# Autodesk Inventor assembly: Ensamblaje2
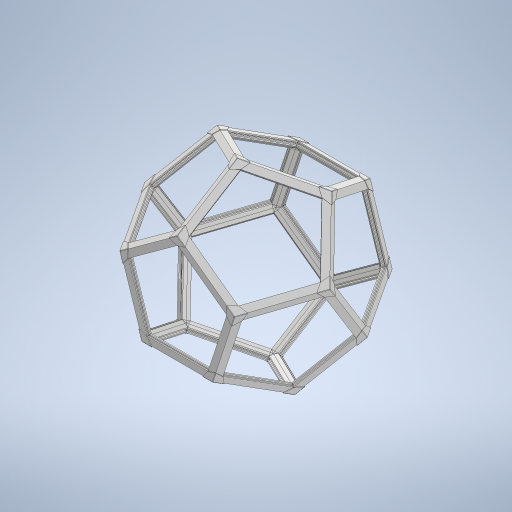
[picture p0: Inventor's stored thumbnail of the model, 512x512]
Saved by Autodesk Inventor 2024 (Build 280153000, 153)
## iProperties
Created: 2025-08-12
Part Number: Ensamblaje2
Document SubType Name: Assembly
Designer: sergi
Author: sergi
## Documents named in this file (3)
- C:\Users\sergi\OneDrive\Escritorio\Ensamblaje2.iam
- C:\Users\sergi\OneDrive\Escritorio\Ensamblaje1.iam
- C:\Users\sergi\OneDrive\Escritorio\Pieza1.ipt
## Components (52 placed, 2 different names)
1. Ensamblaje1:1 [sub-assembly] — Coincidencia:1, Coincidencia:2, Coincidencia:3, Coincidencia:4, Coincidencia:5, Coincidencia:6, Coincidencia:7, Coincidencia:8, Coincidencia:18
2. Pieza1:1 — Coincidencia:1, Coincidencia:2, Coincidencia:3, Coincidencia:15, Coincidencia:16, Coincidencia:17
3. Pieza1:2 — Coincidencia:4, Coincidencia:5, Coincidencia:12, Coincidencia:13, Coincidencia:14, Coincidencia:18
4. Pieza1:3 — Coincidencia:6, Coincidencia:7, Coincidencia:8, Coincidencia:9, Coincidencia:10, Coincidencia:11
5. Ensamblaje1:2 [sub-assembly] — Coincidencia:15, Coincidencia:16, Coincidencia:17, Coincidencia:28, Coincidencia:29, Coincidencia:30, Coincidencia:40, Coincidencia:41, Coincidencia:42
6. Ensamblaje1:3 [sub-assembly] — Coincidencia:9, Coincidencia:10, Coincidencia:11, Coincidencia:52, Coincidencia:53, Coincidencia:54, Coincidencia:64, Coincidencia:65, Coincidencia:66
7. Ensamblaje1:4 [sub-assembly] — Coincidencia:12, Coincidencia:13, Coincidencia:14, Coincidencia:76, Coincidencia:77, Coincidencia:78, Coincidencia:79, Coincidencia:80, Coincidencia:81
8. Ensamblaje1:5 [sub-assembly]
9. Pieza1:4 — Coincidencia:28, Coincidencia:29, Coincidencia:30
10. Pieza1:5
11. Pieza1:6 — Coincidencia:85, Coincidencia:86, Coincidencia:87
12. Ensamblaje1:6 [sub-assembly]
13. Pieza1:7
14. Pieza1:8 — Coincidencia:142, Coincidencia:143, Coincidencia:144
15. Pieza1:9 — Coincidencia:40, Coincidencia:41, Coincidencia:42
16. Ensamblaje1:7 [sub-assembly]
17. Pieza1:11 — Coincidencia:52, Coincidencia:53, Coincidencia:54
18. Pieza1:12
19. Ensamblaje1:8 [sub-assembly]
20. Pieza1:13 — Coincidencia:64, Coincidencia:65, Coincidencia:66
21. Pieza1:14
22. Pieza1:15 — Coincidencia:118, Coincidencia:119, Coincidencia:120
23. Ensamblaje1:9 [sub-assembly]
24. Pieza1:16 — Coincidencia:76, Coincidencia:77, Coincidencia:78
25. Pieza1:17 — Coincidencia:94, Coincidencia:95, Coincidencia:96
26. Pieza1:18 — Coincidencia:79, Coincidencia:80, Coincidencia:81
27. Ensamblaje1:10 [sub-assembly] — Coincidencia:85, Coincidencia:86, Coincidencia:87
28. Pieza1:19
29. Ensamblaje1:11 [sub-assembly] — Coincidencia:103, Coincidencia:104, Coincidencia:105
30. Ensamblaje1:12 [sub-assembly] — Coincidencia:94, Coincidencia:95, Coincidencia:96, Coincidencia:115, Coincidencia:116, Coincidencia:117
31. Pieza1:20
32. Pieza1:22 — Coincidencia:103, Coincidencia:104, Coincidencia:105, Coincidencia:145, Coincidencia:146, Coincidencia:147
33. Ensamblaje1:13 [sub-assembly]
34. Pieza1:23
35. Pieza1:24 — Coincidencia:115, Coincidencia:116, Coincidencia:117
36. Pieza1:25
37. Ensamblaje1:14 [sub-assembly] — Coincidencia:118, Coincidencia:119, Coincidencia:120, Coincidencia:124, Coincidencia:125, Coincidencia:126
38. Ensamblaje1:15 [sub-assembly] — Coincidencia:163, Coincidencia:164, Coincidencia:165
39. Pieza1:26 — Coincidencia:124, Coincidencia:125, Coincidencia:126
40. Ensamblaje1:16 [sub-assembly] — Coincidencia:142, Coincidencia:143, Coincidencia:144, Coincidencia:157, Coincidencia:158, Coincidencia:159
41. Pieza1:27
42. Ensamblaje1:17 [sub-assembly]
43. Ensamblaje1:18 [sub-assembly]
44. Pieza1:28
45. Pieza1:29
46. Ensamblaje1:19 [sub-assembly] — Coincidencia:145, Coincidencia:146, Coincidencia:147, Coincidencia:148, Coincidencia:149, Coincidencia:150
47. Pieza1:30 — Coincidencia:148, Coincidencia:149, Coincidencia:150, Coincidencia:151, Coincidencia:152, Coincidencia:153
48. Ensamblaje1:20 [sub-assembly] — Coincidencia:151, Coincidencia:152, Coincidencia:153
49. Pieza1:31 — Coincidencia:157, Coincidencia:158, Coincidencia:159
50. Ensamblaje1:21 [sub-assembly] — Coincidencia:160, Coincidencia:161, Coincidencia:162
51. Pieza1:32 — Coincidencia:160, Coincidencia:161, Coincidencia:162
52. Pieza1:33 — Coincidencia:163, Coincidencia:164, Coincidencia:165
## Relationships (153: Mate 153)
- Coincidencia:1 [Mate]: Ensamblaje1:1 ↔ Pieza1:1
- Coincidencia:2 [Mate]: Ensamblaje1:1 ↔ Pieza1:1
- Coincidencia:3 [Mate]: Ensamblaje1:1 ↔ Pieza1:1
- Coincidencia:4 [Mate]: Ensamblaje1:1 ↔ Pieza1:2
- Coincidencia:5 [Mate]: Ensamblaje1:1 ↔ Pieza1:2
- Coincidencia:6 [Mate]: Ensamblaje1:1 ↔ Pieza1:3
- Coincidencia:7 [Mate]: Ensamblaje1:1 ↔ Pieza1:3
- Coincidencia:8 [Mate]: Ensamblaje1:1 ↔ Pieza1:3
- Coincidencia:9 [Mate]: Pieza1:3 ↔ Ensamblaje1:3
- Coincidencia:10 [Mate]: Pieza1:3 ↔ Ensamblaje1:3
- Coincidencia:11 [Mate]: Pieza1:3 ↔ Ensamblaje1:3
- Coincidencia:12 [Mate]: Pieza1:2 ↔ Ensamblaje1:4
- Coincidencia:13 [Mate]: Pieza1:2 ↔ Ensamblaje1:4
- Coincidencia:14 [Mate]: Pieza1:2 ↔ Ensamblaje1:4
- Coincidencia:15 [Mate]: Pieza1:1 ↔ Ensamblaje1:2
- Coincidencia:16 [Mate]: Pieza1:1 ↔ Ensamblaje1:2
- Coincidencia:17 [Mate]: Pieza1:1 ↔ Ensamblaje1:2
- Coincidencia:18 [Mate]: Ensamblaje1:1 ↔ Pieza1:2
- [Mate]: Ensamblaje1:5 ↔ Pieza1:4
- [Mate]: Ensamblaje1:5 ↔ Pieza1:4
- [Mate]: Ensamblaje1:5 ↔ Pieza1:4
- [Mate]: Ensamblaje1:5 ↔ Pieza1:5
- [Mate]: Ensamblaje1:5 ↔ Pieza1:5
- [Mate]: Ensamblaje1:5 ↔ Pieza1:6
- [Mate]: Ensamblaje1:5 ↔ Pieza1:6
- [Mate]: Ensamblaje1:5 ↔ Pieza1:6
- [Mate]: Ensamblaje1:5 ↔ Pieza1:5
- Coincidencia:28 [Mate]: Ensamblaje1:2 ↔ Pieza1:4
- Coincidencia:29 [Mate]: Ensamblaje1:2 ↔ Pieza1:4
- Coincidencia:30 [Mate]: Ensamblaje1:2 ↔ Pieza1:4
- [Mate]: Ensamblaje1:6 ↔ Pieza1:7
- [Mate]: Ensamblaje1:6 ↔ Pieza1:7
- [Mate]: Ensamblaje1:6 ↔ Pieza1:7
- [Mate]: Ensamblaje1:6 ↔ Pieza1:8
- [Mate]: Ensamblaje1:6 ↔ Pieza1:8
- [Mate]: Ensamblaje1:6 ↔ Pieza1:9
- [Mate]: Ensamblaje1:6 ↔ Pieza1:9
- [Mate]: Ensamblaje1:6 ↔ Pieza1:9
- [Mate]: Ensamblaje1:6 ↔ Pieza1:8
- Coincidencia:40 [Mate]: Ensamblaje1:2 ↔ Pieza1:9
- Coincidencia:41 [Mate]: Ensamblaje1:2 ↔ Pieza1:9
- Coincidencia:42 [Mate]: Ensamblaje1:2 ↔ Pieza1:9
- [Mate]: Ensamblaje1:7 ↔ Pieza1:11
- [Mate]: Ensamblaje1:7 ↔ Pieza1:11
- [Mate]: Ensamblaje1:7 ↔ Pieza1:12
- [Mate]: Ensamblaje1:7 ↔ Pieza1:12
- [Mate]: Ensamblaje1:7 ↔ Pieza1:12
- [Mate]: Ensamblaje1:7 ↔ Pieza1:11
- Coincidencia:52 [Mate]: Ensamblaje1:3 ↔ Pieza1:11
- Coincidencia:53 [Mate]: Ensamblaje1:3 ↔ Pieza1:11
- Coincidencia:54 [Mate]: Ensamblaje1:3 ↔ Pieza1:11
- [Mate]: Ensamblaje1:8 ↔ Pieza1:13
- [Mate]: Ensamblaje1:8 ↔ Pieza1:13
- [Mate]: Ensamblaje1:8 ↔ Pieza1:13
- [Mate]: Ensamblaje1:8 ↔ Pieza1:14
- [Mate]: Ensamblaje1:8 ↔ Pieza1:14
- [Mate]: Ensamblaje1:8 ↔ Pieza1:15
- [Mate]: Ensamblaje1:8 ↔ Pieza1:15
- [Mate]: Ensamblaje1:8 ↔ Pieza1:15
- [Mate]: Ensamblaje1:8 ↔ Pieza1:14
- Coincidencia:64 [Mate]: Ensamblaje1:3 ↔ Pieza1:13
- Coincidencia:65 [Mate]: Ensamblaje1:3 ↔ Pieza1:13
- Coincidencia:66 [Mate]: Ensamblaje1:3 ↔ Pieza1:13
- [Mate]: Ensamblaje1:9 ↔ Pieza1:16
- [Mate]: Ensamblaje1:9 ↔ Pieza1:16
- [Mate]: Ensamblaje1:9 ↔ Pieza1:16
- [Mate]: Ensamblaje1:9 ↔ Pieza1:17
- [Mate]: Ensamblaje1:9 ↔ Pieza1:17
- [Mate]: Ensamblaje1:9 ↔ Pieza1:17
- Coincidencia:76 [Mate]: Ensamblaje1:4 ↔ Pieza1:16
- Coincidencia:77 [Mate]: Ensamblaje1:4 ↔ Pieza1:16
- Coincidencia:78 [Mate]: Ensamblaje1:4 ↔ Pieza1:16
- Coincidencia:79 [Mate]: Ensamblaje1:4 ↔ Pieza1:18
- Coincidencia:80 [Mate]: Ensamblaje1:4 ↔ Pieza1:18
- Coincidencia:81 [Mate]: Ensamblaje1:4 ↔ Pieza1:18
- [Mate]: Ensamblaje1:10 ↔ Pieza1:19
- [Mate]: Ensamblaje1:10 ↔ Pieza1:19
- [Mate]: Ensamblaje1:10 ↔ Pieza1:19
- Coincidencia:85 [Mate]: Pieza1:6 ↔ Ensamblaje1:10
- Coincidencia:86 [Mate]: Pieza1:6 ↔ Ensamblaje1:10
- Coincidencia:87 [Mate]: Pieza1:6 ↔ Ensamblaje1:10
- [Mate]: Ensamblaje1:12 ↔ Pieza1:20
- [Mate]: Ensamblaje1:12 ↔ Pieza1:20
- [Mate]: Ensamblaje1:12 ↔ Pieza1:20
- [Mate]: Ensamblaje1:11 ↔ Pieza1:20
- [Mate]: Ensamblaje1:11 ↔ Pieza1:20
- [Mate]: Ensamblaje1:11 ↔ Pieza1:20
- Coincidencia:94 [Mate]: Pieza1:17 ↔ Ensamblaje1:12
- Coincidencia:95 [Mate]: Pieza1:17 ↔ Ensamblaje1:12
- Coincidencia:96 [Mate]: Pieza1:17 ↔ Ensamblaje1:12
- Coincidencia:103 [Mate]: Ensamblaje1:11 ↔ Pieza1:22
- Coincidencia:104 [Mate]: Ensamblaje1:11 ↔ Pieza1:22
- Coincidencia:105 [Mate]: Ensamblaje1:11 ↔ Pieza1:22
- [Mate]: Ensamblaje1:13 ↔ Pieza1:23
- [Mate]: Ensamblaje1:13 ↔ Pieza1:23
- [Mate]: Ensamblaje1:13 ↔ Pieza1:23
- [Mate]: Ensamblaje1:13 ↔ Pieza1:24
- [Mate]: Ensamblaje1:13 ↔ Pieza1:24
- [Mate]: Ensamblaje1:13 ↔ Pieza1:25
- [Mate]: Ensamblaje1:13 ↔ Pieza1:25
- [Mate]: Ensamblaje1:13 ↔ Pieza1:25
- [Mate]: Ensamblaje1:13 ↔ Pieza1:24
- Coincidencia:115 [Mate]: Ensamblaje1:12 ↔ Pieza1:24
- Coincidencia:116 [Mate]: Ensamblaje1:12 ↔ Pieza1:24
- Coincidencia:117 [Mate]: Ensamblaje1:12 ↔ Pieza1:24
- Coincidencia:118 [Mate]: Pieza1:15 ↔ Ensamblaje1:14
- Coincidencia:119 [Mate]: Pieza1:15 ↔ Ensamblaje1:14
- Coincidencia:120 [Mate]: Pieza1:15 ↔ Ensamblaje1:14
- [Mate]: Ensamblaje1:15 ↔ Pieza1:26
- [Mate]: Ensamblaje1:15 ↔ Pieza1:26
- [Mate]: Ensamblaje1:15 ↔ Pieza1:26
- Coincidencia:124 [Mate]: Ensamblaje1:14 ↔ Pieza1:26
- Coincidencia:125 [Mate]: Ensamblaje1:14 ↔ Pieza1:26
- Coincidencia:126 [Mate]: Ensamblaje1:14 ↔ Pieza1:26
- [Mate]: Ensamblaje1:16 ↔ Pieza1:27
- [Mate]: Ensamblaje1:16 ↔ Pieza1:27
- [Mate]: Pieza1:27 ↔ Ensamblaje1:17
- [Mate]: Pieza1:27 ↔ Ensamblaje1:17
- [Mate]: Pieza1:27 ↔ Ensamblaje1:17
- [Mate]: Ensamblaje1:16 ↔ Pieza1:27
- [Mate]: Ensamblaje1:18 ↔ Pieza1:28
- [Mate]: Ensamblaje1:18 ↔ Pieza1:28
- [Mate]: Ensamblaje1:18 ↔ Pieza1:28
- [Mate]: Ensamblaje1:17 ↔ Pieza1:28
- [Mate]: Ensamblaje1:17 ↔ Pieza1:28
- [Mate]: Ensamblaje1:17 ↔ Pieza1:28
- [Mate]: Ensamblaje1:17 ↔ Pieza1:29
- [Mate]: Ensamblaje1:17 ↔ Pieza1:29
- [Mate]: Ensamblaje1:17 ↔ Pieza1:29
- Coincidencia:142 [Mate]: Pieza1:8 ↔ Ensamblaje1:16
- Coincidencia:143 [Mate]: Pieza1:8 ↔ Ensamblaje1:16
- Coincidencia:144 [Mate]: Pieza1:8 ↔ Ensamblaje1:16
- Coincidencia:145 [Mate]: Pieza1:22 ↔ Ensamblaje1:19
- Coincidencia:146 [Mate]: Pieza1:22 ↔ Ensamblaje1:19
- Coincidencia:147 [Mate]: Pieza1:22 ↔ Ensamblaje1:19
- Coincidencia:148 [Mate]: Ensamblaje1:19 ↔ Pieza1:30
- Coincidencia:149 [Mate]: Ensamblaje1:19 ↔ Pieza1:30
- Coincidencia:150 [Mate]: Ensamblaje1:19 ↔ Pieza1:30
- Coincidencia:151 [Mate]: Pieza1:30 ↔ Ensamblaje1:20
- Coincidencia:152 [Mate]: Pieza1:30 ↔ Ensamblaje1:20
- Coincidencia:153 [Mate]: Pieza1:30 ↔ Ensamblaje1:20
- [Mate]: Pieza1:31 ↔ Ensamblaje1:21
- [Mate]: Pieza1:31 ↔ Ensamblaje1:21
- [Mate]: Pieza1:31 ↔ Ensamblaje1:21
- Coincidencia:157 [Mate]: Ensamblaje1:16 ↔ Pieza1:31
- Coincidencia:158 [Mate]: Ensamblaje1:16 ↔ Pieza1:31
- Coincidencia:159 [Mate]: Ensamblaje1:16 ↔ Pieza1:31
- Coincidencia:160 [Mate]: Ensamblaje1:21 ↔ Pieza1:32
- Coincidencia:161 [Mate]: Ensamblaje1:21 ↔ Pieza1:32
- Coincidencia:162 [Mate]: Ensamblaje1:21 ↔ Pieza1:32
- Coincidencia:163 [Mate]: Ensamblaje1:15 ↔ Pieza1:33
- Coincidencia:164 [Mate]: Ensamblaje1:15 ↔ Pieza1:33
- Coincidencia:165 [Mate]: Ensamblaje1:15 ↔ Pieza1:33
## Named parameters: d18_d17 = 0 mm, d19_d2 = 0 mm, d20_d3 = 0 mm, d21_d4 = 0 mm, d22_d5 = 0 mm, d23_d6 = 0 mm, d24_d7 = 0 mm, d25_d0 = 0 mm, d26_d1 = 0 mm, d30_d17 = 0 mm, d31_d2 = 0 mm, d32_d3 = 0 mm, d33_d4 = 0 mm, d34_d5 = 0 mm, d35_d6 = 0 mm, d36_d7 = 0 mm, d37_d0 = 0 mm, d38_d1 = 0 mm, d42_d17 = 0 mm, d44_d3 = 0 mm, d45_d4 = 0 mm, d46_d5 = 0 mm, d47_d6 = 0 mm, d48_d7 = 0 mm, d54_d17 = 0 mm, d55_d2 = 0 mm, d56_d3 = 0 mm, d57_d4 = 0 mm, d58_d5 = 0 mm, d59_d6 = 0 mm, d60_d7 = 0 mm, d61_d0 = 0 mm, d62_d1 = 0 mm, d66_d17 = 0 mm, d67_d2 = 0 mm, d68_d3 = 0 mm, d69_d4 = 0 mm, d73_d0 = 0 mm, d74_d1 = 0 mm, d81_d66_d17 = 0 mm, d82_d68_d3 = 0 mm, d83_d69_d4 = 0 mm, d87_d67_d2 = 0 mm, d88_d73_d0 = 0 mm, d89_d74_d1 = 0 mm, d90_d75 = 0 mm, d91_d76 = 0 mm, d92_d77 = 0 mm, d105_d17 = 0 mm, d106_d2 = 0 mm, d107_d3 = 0 mm, d108_d4 = 0 mm, d109_d5 = 0 mm, d110_d6 = 0 mm, d111_d7 = 0 mm, d112_d0 = 0 mm, d113_d1 = 0 mm, d120_d109_d5 = 0 mm, d121_d110_d6 = 0 mm, d122_d111_d7 = 0 mm, d126_d13 = 0 mm, d127_d17 = 0 mm, d128_d3 = 0 mm, d129_d4 = 0 mm, d130_d11 = 0 mm, d131_d12 = 0 mm, d132_d80 = 0 mm, d133_d67_d2 = 0 mm, d134_d73_d0 = 0 mm, d135_d74_d1 = 0 mm, d136_d75 = 0 mm, d137_d76 = 0 mm, d138_d77 = 0 mm, d139_d78 = 0 mm, d140_d79 = 0 mm, d153_d141 = 0 mm, d154_d142 = 0 mm, d155_d143 = 0 mm
